# Autodesk Inventor assembly: Assembly1
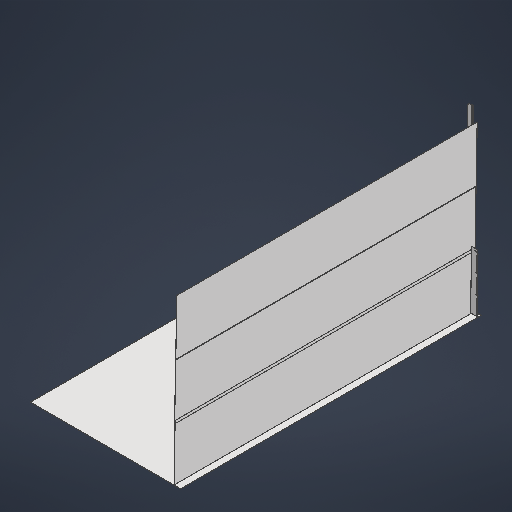
[picture p0: Inventor's stored thumbnail of the model, 512x512]
Saved by Autodesk Inventor 2026.2 (Build 302298000, 298)
## iProperties
Created: 2026-04-17
Part Number: Assembly1
Document SubType Name: Assembly
Designer: admin
Author: admin
## Documents named in this file (6)
- C:\Users\admin\Documents\Inventor\GBK-Gubkinskiy\Assembly1.iam
- C:\Users\admin\Documents\Inventor\GBK-Gubkinskiy\Part1.ipt
- C:\Users\admin\Documents\Inventor\GBK-Gubkinskiy\Part2.ipt
- C:\Users\admin\Documents\Inventor\GBK-Gubkinskiy\Part2_CPY.ipt
- C:\Users\admin\Documents\Inventor\GBK-Gubkinskiy\Part2_CPY_CPY.ipt
- C:\Users\admin\Documents\Inventor\GBK-Gubkinskiy\Part111.ipt
## Components (7 placed, 5 different names)
1. Part1:1 — Rigid:1, Flush:1, Mate:4
2. Part111:1 — Flush:1, Mate:3, Mate:4, Mate:5
3. Part111:2 — Flush:2, Mate:5, Mate:6, Flush:3
4. Part111:3 — Mate:6, Flush:3
5. Part2_CPY_CPY:1 — Rigid:3
6. Part2_CPY:1 — Rigid:2, Rigid:3, Flush:2
7. Part2:1 — Rigid:1, Rigid:2, Mate:3
## Relationships (10: Mate 4, WeldJoint 3, Flush 3)
- Rigid:1 [WeldJoint]: Part1:1 ↔ Part2:1
- Rigid:2 [WeldJoint] (-50 mm): Part2_CPY:1 ↔ Part2:1
- Rigid:3 [WeldJoint] (-50 mm): Part2_CPY_CPY:1 ↔ Part2_CPY:1
- Flush:1: Part1:1 ↔ Part111:1
- Mate:3: Part111:1 ↔ Part2:1
- Mate:4: Part1:1 ↔ Part111:1
- Flush:2: Part111:2 ↔ Part2_CPY:1
- Mate:5: Part111:1 ↔ Part111:2
- Mate:6: Part111:2 ↔ Part111:3
- Flush:3: Part111:2 ↔ Part111:3
